# Autodesk Inventor assembly: appereture
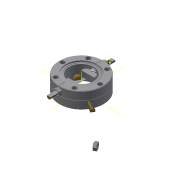
[picture p0: Inventor's stored thumbnail of the model, 180x180]
Saved by Autodesk Inventor 2015 (Build 190159000, 159)
## iProperties
Created: 2015-10-28
Part Number: appereture
Document SubType Name: Assembly
Designer: jad211
Author: jad211
## Documents named in this file (7)
- C:\CADFiles\Adjustable apperture\appereture.iam
- C:\CADFiles\Adjustable apperture\Flange.ipt
- C:\CADFiles\Adjustable apperture\rod.ipt
- C:\CADFiles\Adjustable apperture\m2 bolt.ipt
- C:\CADFiles\Adjustable apperture\m6nut.ipt
- C:\CADFiles\Adjustable apperture\bladefull.ipt
- C:\CADFiles\Adjustable apperture\bladehalf.ipt
## Components (17 placed, 6 different names)
1. Flange:1 — Mate:1, Angle:1, Mate:2, Mate:3, Angle:3, Angle:4, Angle:5, Mate:9, Mate:10, Mate:11, Angle:8, Mate:29, Flush:1, Flush:2, Mate:30, Mate:31, Mate:32
2. rod:1 — Mate:1, Angle:1, Mate:7, Mate:12, Mate:17, Angle:6
3. rod:2 — Mate:2, Angle:5, Mate:6, Mate:14, Mate:19, Angle:7
4. rod:3 — Mate:3, Angle:3, Mate:15, Mate:22, Mate:26, Mate:28
5. rod:4 — Angle:4, Mate:23, Mate:25, Mate:32
6. m2 bolt:1 — Mate:23, Mate:24
7. m2 bolt:2 — Mate:7, Mate:16, Mate:21
8. m2 bolt:3 — Mate:22, Mate:27
9. m2 bolt:4 — Mate:6, Mate:18, Mate:20
10. m6nut:1 — Mate:12, Flush:1
11. m6nut:2 — Mate:15, Flush:2
12. m6nut:3 — Mate:29, Mate:30
13. m6nut:4 — Mate:14, Mate:31
14. bladefull:1 — Mate:16, Mate:17, Angle:6, Mate:21
15. bladefull:2 — Mate:18, Mate:19, Angle:7, Mate:20
16. bladehalf:1 — Mate:24, Mate:25, Angle:8
17. bladehalf:2 — Mate:26, Mate:27, Mate:28, Angle:9
## Relationships (38: Mate 28, Angle 8, Flush 2)
- Mate:1: Flange:1 ↔ rod:1
- Angle:1 (0 deg): Flange:1 ↔ rod:1
- Mate:2: Flange:1 ↔ rod:2
- Mate:3: Flange:1 ↔ rod:3
- Angle:3 (180 deg): Flange:1 ↔ rod:3
- Angle:4 (180 deg): Flange:1 ↔ rod:4
- Angle:5 (0 deg): Flange:1 ↔ rod:2
- Mate:6: rod:2 ↔ m2 bolt:4
- Mate:7: rod:1 ↔ m2 bolt:2
- Mate:9: Flange:1
- Mate:10: Flange:1
- Mate:11: Flange:1
- Mate:12: rod:1 ↔ m6nut:1
- Mate:14: rod:2 ↔ m6nut:4
- Mate:15: rod:3 ↔ m6nut:2
- Mate:16: m2 bolt:2 ↔ bladefull:1
- Mate:17: rod:1 ↔ bladefull:1
- Angle:6 (0 deg): rod:1 ↔ bladefull:1
- Mate:18: m2 bolt:4 ↔ bladefull:2
- Mate:19: rod:2 ↔ bladefull:2
- Angle:7 (0 deg): rod:2 ↔ bladefull:2
- Mate:20: m2 bolt:4 ↔ bladefull:2
- Mate:21: m2 bolt:2 ↔ bladefull:1
- Mate:22: rod:3 ↔ m2 bolt:3
- Mate:23: rod:4 ↔ m2 bolt:1
- Mate:24: m2 bolt:1 ↔ bladehalf:1
- Mate:25: rod:4 ↔ bladehalf:1
- Angle:8 (180 deg): Flange:1 ↔ bladehalf:1
- Mate:26: rod:3 ↔ bladehalf:2
- Mate:27: m2 bolt:3 ↔ bladehalf:2
- Mate:28: rod:3 ↔ bladehalf:2
- Angle:9 (0 deg): bladehalf:2
- Mate:29: Flange:1 ↔ m6nut:3
- Flush:1: Flange:1 ↔ m6nut:1
- Flush:2: Flange:1 ↔ m6nut:2
- Mate:30: Flange:1 ↔ m6nut:3
- Mate:31: Flange:1 ↔ m6nut:4
- Mate:32: Flange:1 ↔ rod:4
